# Autodesk Inventor assembly: złożenie_690
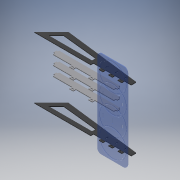
[picture p0: Inventor's stored thumbnail of the model, 180x180]
Saved by Autodesk Inventor 2017 (Build 210142000, 142)
## iProperties
Part Number: złożenie_690
Material: Ogólny
Document SubType Name: Assembly
Designer: patry
Author: patry
## Documents named in this file (4)
- C:\Users\patry\Desktop\Mocowanie_wykrywacz\złożenie_690.iam
- C:\Users\patry\Desktop\Mocowanie_wykrywacz\bok.ipt
- C:\Users\patry\Desktop\Mocowanie_wykrywacz\Cewki_690.ipt
- C:\Users\patry\Desktop\Mocowanie_wykrywacz\poprz_690.ipt
## Components (6 placed, 3 different names)
1. bok:1 — Zestawiający:2, Zestawiający:3, Zestawiający:6
2. Cewki_690:1 — Zestawiający:1, Zestawiający:2, Zestawiający:3, Zestawiający:4, Zestawiający:5, Zestawiający:6, Zestawiający:7
3. bok:2 — Zestawiający:1, Zestawiający:4, Zestawiający:5
4. poprz_690:1 — Równoległy:1, Równoległy:3, Równoległy:4, Równoległy:5
5. poprz_690:2 — Równoległy:1, Równoległy:2, Równoległy:3, Równoległy:5, Równoległy:6, Zestawiający:7
6. poprz_690:3 — Równoległy:2, Równoległy:4, Równoległy:6
## Relationships (13: Mate 7, Flush 6)
- Zestawiający:1 [Mate]: Cewki_690:1 ↔ bok:2
- Zestawiający:2 [Mate]: bok:1 ↔ Cewki_690:1
- Zestawiający:3 [Mate]: bok:1 ↔ Cewki_690:1
- Zestawiający:4 [Mate]: Cewki_690:1 ↔ bok:2
- Zestawiający:5 [Mate]: Cewki_690:1 ↔ bok:2
- Zestawiający:6 [Mate]: bok:1 ↔ Cewki_690:1
- Równoległy:1 [Flush]: poprz_690:1 ↔ poprz_690:2
- Równoległy:2 [Flush]: poprz_690:2 ↔ poprz_690:3
- Równoległy:3 [Flush]: poprz_690:1 ↔ poprz_690:2
- Równoległy:4 [Flush]: poprz_690:1 ↔ poprz_690:3
- Równoległy:5 [Flush] (70 mm): poprz_690:1 ↔ poprz_690:2
- Równoległy:6 [Flush] (70 mm): poprz_690:2 ↔ poprz_690:3
- Zestawiający:7 [Mate]: Cewki_690:1 ↔ poprz_690:2
